# Autodesk Inventor assembly: Assembly1
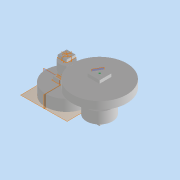
[picture p0: Inventor's stored thumbnail of the model, 180x180]
Saved by Autodesk Inventor 2022 (Build 260153000, 153)
## iProperties
Created: 2024-01-11
Part Number: Assembly1
Document SubType Name: Assembly
Designer: ktamu
Author: ktamu
## Documents named in this file (11)
- D:\SDinventor\InventTryagainInvo\Assembly1.iam
- D:\SDinventor\InventTryagainInvo\bearing1b.ipt
- D:\SDinventor\InventTryagainInvo\gear1.ipt
- D:\SDinventor\InventTryagainInvo\shaft1.ipt
- D:\SDinventor\InventTryagainInvo\bearing2b.ipt
- D:\SDinventor\InventTryagainInvo\shift2.ipt
- D:\SDinventor\InventTryagainInvo\gear2.ipt
- D:\SDinventor\InventTryagainInvo\gear3.ipt
- D:\SDinventor\InventTryagainInvo\bearing3b.ipt
- D:\SDinventor\InventTryagainInvo\shaft3.ipt
- C:\Users\Public\Documents\Autodesk\.desktop-connect\.docstore\guided-tutorial-plugin\INVNTOR\2018\ENU\904018470784649253\TutorialModelPath\0\gear4.ipt
## Components (13 placed, 10 different names)
1. bearing1b:1 — フラッシュ:1, フラッシュ:2, フラッシュ:3, メイト:7, メイト:8
2. bearing1b:2 — フラッシュ:1, フラッシュ:2, フラッシュ:3, 回転:1, メイト:1, メイト:3, フラッシュ:5, メイト:4, メイト:9
3. gear1:1 — メイト:7, 回転:3, フラッシュ:7
4. shaft1:1 — 回転:1, 回転:3, フラッシュ:7, 回転:2
5. bearing2b:1 — メイト:2, フラッシュ:5, メイト:4, メイト:5, メイト:6, フラッシュ:6
6. bearing2b:2 — メイト:1, メイト:2, メイト:3, メイト:5, メイト:6, 角度:1, 回転:2, フラッシュ:9, フラッシュ:11
7. shift2:1 — 角度:1, 回転:2, 回転:4, フラッシュ:8, 回転:5, フラッシュ:10, 回転:1, 回転:2
8. gear2:1 — フラッシュ:6, 回転:4, フラッシュ:8
9. gear3:1 — フラッシュ:9, 回転:5, フラッシュ:10
10. bearing3b:1 — フラッシュ:11, メイト:8, メイト:9, フラッシュ:12, メイト:10, メイト:11, 回転:6
11. bearing3b:2 — フラッシュ:12, メイト:10, メイト:11
12. shaft3:1 — 回転:6, 回転:7, フラッシュ:13, 回転:1
13. gear4:1 — 回転:7, フラッシュ:13
## Relationships (33: Flush 12, Mate 11, RevoluteJoint 7, RelateRotation 2, Angle 1)
- フラッシュ:1 [Flush]: bearing1b:1 ↔ bearing1b:2
- フラッシュ:2 [Flush]: bearing1b:1 ↔ bearing1b:2
- フラッシュ:3 [Flush] (77 mm): bearing1b:1 ↔ bearing1b:2
- 回転:1 [RevoluteJoint]: bearing1b:2 ↔ shaft1:1
- メイト:1 [Mate]: bearing1b:2 ↔ bearing2b:2
- メイト:2 [Mate]: bearing2b:1 ↔ bearing2b:2
- メイト:3 [Mate]: bearing1b:2 ↔ bearing2b:2
- フラッシュ:5 [Flush]: bearing1b:2 ↔ bearing2b:1
- メイト:4 [Mate] (174 mm): bearing1b:2 ↔ bearing2b:1
- メイト:5 [Mate] (-210 mm): bearing2b:1 ↔ bearing2b:2
- メイト:6 [Mate]: bearing2b:1 ↔ bearing2b:2
- 角度:1 [Angle] (180 deg): bearing2b:2 ↔ shift2:1
- 回転:2 [RevoluteJoint]: bearing2b:2 ↔ shift2:1
- フラッシュ:6 [Flush] (25 mm): bearing2b:1 ↔ gear2:1
- メイト:7 [Mate] (-25 mm): bearing1b:1 ↔ gear1:1
- 回転:3 [RevoluteJoint] (-25 mm): gear1:1 ↔ shaft1:1
- フラッシュ:7 [Flush]: gear1:1 ↔ shaft1:1
- 回転:4 [RevoluteJoint] (25 mm): shift2:1 ↔ gear2:1
- フラッシュ:8 [Flush]: shift2:1 ↔ gear2:1
- フラッシュ:9 [Flush] (25 mm): bearing2b:2 ↔ gear3:1
- 回転:5 [RevoluteJoint] (-25 mm): shift2:1 ↔ gear3:1
- フラッシュ:10 [Flush]: shift2:1 ↔ gear3:1
- フラッシュ:11 [Flush]: bearing2b:2 ↔ bearing3b:1
- メイト:8 [Mate]: bearing1b:1 ↔ bearing3b:1
- メイト:9 [Mate] (-210 mm): bearing1b:2 ↔ bearing3b:1
- フラッシュ:12 [Flush]: bearing3b:1 ↔ bearing3b:2
- メイト:10 [Mate]: bearing3b:1 ↔ bearing3b:2
- メイト:11 [Mate] (-110 mm): bearing3b:1 ↔ bearing3b:2
- 回転:6 [RevoluteJoint]: bearing3b:1 ↔ shaft3:1
- 回転:7 [RevoluteJoint] (-25 mm): shaft3:1 ↔ gear4:1
- フラッシュ:13 [Flush]: shaft3:1 ↔ gear4:1
- 回転:1 [RelateRotation] (4.1177 ul): shift2:1 ↔ shaft3:1
- 回転:2 [RelateRotation] (0.5675 ul): shaft1:1 ↔ shift2:1
